# Autodesk Inventor assembly: Control Cabinet Unit
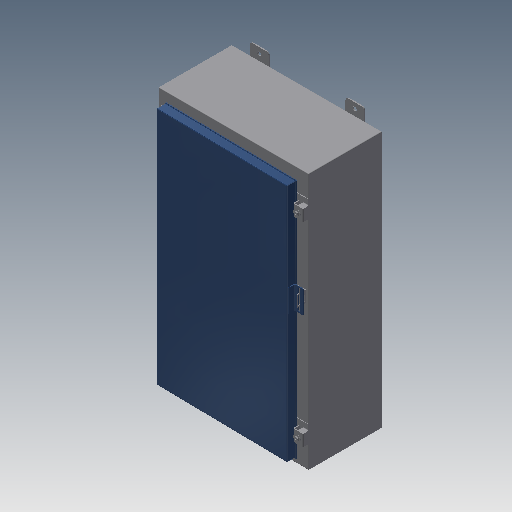
[picture p0: Inventor's stored thumbnail of the model, 512x512]
Saved by Autodesk Inventor 2020 (Build 240152000, 152)
## iProperties
Created: 2006-09-21
Part Number: Control Cabinet Unit
Document SubType Name: Assembly
Designer: floress
Description: Separator PLC Controller
Stock Number: NA
Mass: 3685.2 g
Surface Area: 40299.7 cm^2
Volume: 3667.4 cm^3
Density: 1.00485 g/cm^3
Author: floress
Title: In House Assembly
Revision Number: A
## Documents named in this file (6)
- C:\Users\hallc\Desktop\Process Equipment\Workspace\Components\Control Cabinet Unit.iam
- C:\Users\hallc\Desktop\Process Equipment\Workspace\Supplier Content\Electrical Design\PC Case\PC Case.iam
- C:\Users\hallc\Desktop\Process Equipment\Workspace\Supplier Content\Electrical Design\Motherboard\Motherboard.iam
- C:\Users\hallc\Desktop\Process Equipment\Workspace\Supplier Content\Electrical Design\Graphics Card\Graphics Card.iam
- C:\Users\hallc\Desktop\Process Equipment\Workspace\Supplier Content\Electrical Design\Power Supply\Power Supply.iam
- C:\Users\hallc\Desktop\Process Equipment\Workspace\Supplier Content\Electrical Design\Single Door Enclosure\PLC Casing Enclosure.iam
## Components (5 placed, 5 different names)
1. PC Case:1 [sub-assembly] — Mate:3, Flush:1, Mate:4, Mate:8, Mate:1, Flush:11, Flush:12, Mate:110, Mate:112
2. Power Supply:1 [sub-assembly] — Mate:8, Flush:11
3. Motherboard:1 [sub-assembly] — Mate:2, Mate:5, Mate:1, Flush:12
4. Graphics Card:1 [sub-assembly] — Mate:2, Mate:3, Flush:1, Mate:4, Mate:5
5. PLC Casing Enclosure:1 [sub-assembly] — Mate:110, Mate:112
## Relationships (11: Mate 8, Flush 3)
- Mate:2: Motherboard:1 ↔ Graphics Card:1
- Mate:3: PC Case:1 ↔ Graphics Card:1
- Flush:1 (21.4884 mm): PC Case:1 ↔ Graphics Card:1
- Mate:4: PC Case:1 ↔ Graphics Card:1
- Mate:5: Motherboard:1 ↔ Graphics Card:1
- Mate:8: PC Case:1 ↔ Power Supply:1
- Mate:1: PC Case:1 ↔ Motherboard:1
- Flush:11: PC Case:1 ↔ Power Supply:1
- Flush:12 (-14 mm): PC Case:1 ↔ Motherboard:1
- Mate:110: PC Case:1 ↔ PLC Casing Enclosure:1
- Mate:112: PC Case:1 ↔ PLC Casing Enclosure:1
